# Autodesk Inventor assembly: Front Hitch Model-2
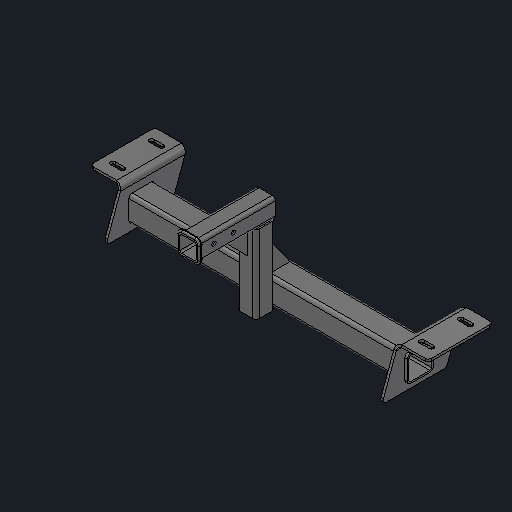
[picture p0: Inventor's stored thumbnail of the model, 512x512]
Saved by Autodesk Inventor 2025.1 (Build 291241000, 241)
## iProperties
Created: 2026-02-13
Part Number: Front Hitch Model-2
Document SubType Name: Assembly
Designer: Desktop -24
encoded128: ÌStandard (in)rÎ
Family: ASSEMBLY
Author: Desktop -24
## Documents named in this file (8)
- F:\OneDrive - nLeague Technologies Private Limited\Desktop\Sharath Chandra\Front Hitch\Front Hitch Model-2\Front Hitch Model-2.iam
- F:\OneDrive - nLeague Technologies Private Limited\Desktop\Sharath Chandra\Front Hitch\Front Hitch Model-1\Front Hitch Model-1_Base Tube-2.ipt
- F:\OneDrive - nLeague Technologies Private Limited\Desktop\Sharath Chandra\Front Hitch\Front Hitch Model-2\Front Hitch Model-2_Base Tube-1.ipt
- F:\OneDrive - nLeague Technologies Private Limited\Desktop\Sharath Chandra\Front Hitch\Front Hitch Model-2\Front Hitch Model-1_Base Tube-3.ipt
- F:\OneDrive - nLeague Technologies Private Limited\Desktop\Sharath Chandra\Front Hitch\Front Hitch Model-2\Front Hitch Model-2_Sheet Stifferner-1.ipt
- F:\OneDrive - nLeague Technologies Private Limited\Desktop\Sharath Chandra\Front Hitch\Front Hitch Model-2\Front Hitch Model-2_Sheet Stifferner-2.ipt
- F:\OneDrive - nLeague Technologies Private Limited\Desktop\Sharath Chandra\Front Hitch\Front Hitch Model-2\Front Hitch Model-2_Sheet-RH.ipt
- F:\OneDrive - nLeague Technologies Private Limited\Desktop\Sharath Chandra\Front Hitch\Front Hitch Model-2\Front Hitch Model-2_Sheet-LH.ipt
## Components (7 placed, 7 different names)
1. Front Hitch Model-2_Base Tube-1.ipt:1 — Mate:14, Mate:15, Mate:16, Mate:17, Mate:18, Flush:8, Flush:9, Flush:12, Mate:20, Mate:21, Mate:23
2. Front Hitch Model-2_Sheet-LH.ipt:1 — Mate:17, Mate:18, Flush:8
3. Front Hitch Model-2_Sheet-RH.ipt:1 — Mate:15, Mate:16, Flush:9
4. Front Hitch Model-1_Base Tube-2.ipt:1 — Mate:19, Flush:10, Flush:11, Mate:25
5. Front Hitch Model-1_Base Tube-3.ipt:1 — Mate:19, Flush:10, Flush:11, Flush:12, Mate:20, Mate:21, Mate:22, Mate:24
6. Front Hitch Model-2_Sheet Stifferner-2.ipt:1 — Mate:22, Mate:23
7. Front Hitch Model-2_Sheet Stifferner-1.ipt:1 — Mate:24, Mate:25
## Relationships (17: Mate 12, Flush 5)
- Mate:14: Front Hitch Model-2_Base Tube-1.ipt:1
- Mate:15: Front Hitch Model-2_Base Tube-1.ipt:1 ↔ Front Hitch Model-2_Sheet-RH.ipt:1
- Mate:16: Front Hitch Model-2_Base Tube-1.ipt:1 ↔ Front Hitch Model-2_Sheet-RH.ipt:1
- Mate:17: Front Hitch Model-2_Base Tube-1.ipt:1 ↔ Front Hitch Model-2_Sheet-LH.ipt:1
- Mate:18: Front Hitch Model-2_Base Tube-1.ipt:1 ↔ Front Hitch Model-2_Sheet-LH.ipt:1
- Flush:8 (9.525 mm): Front Hitch Model-2_Base Tube-1.ipt:1 ↔ Front Hitch Model-2_Sheet-LH.ipt:1
- Flush:9 (-9.525 mm): Front Hitch Model-2_Base Tube-1.ipt:1 ↔ Front Hitch Model-2_Sheet-RH.ipt:1
- Mate:19: Front Hitch Model-1_Base Tube-2.ipt:1 ↔ Front Hitch Model-1_Base Tube-3.ipt:1
- Flush:10: Front Hitch Model-1_Base Tube-2.ipt:1 ↔ Front Hitch Model-1_Base Tube-3.ipt:1
- Flush:11: Front Hitch Model-1_Base Tube-2.ipt:1 ↔ Front Hitch Model-1_Base Tube-3.ipt:1
- Flush:12: Front Hitch Model-2_Base Tube-1.ipt:1 ↔ Front Hitch Model-1_Base Tube-3.ipt:1
- Mate:20: Front Hitch Model-2_Base Tube-1.ipt:1 ↔ Front Hitch Model-1_Base Tube-3.ipt:1
- Mate:21: Front Hitch Model-2_Base Tube-1.ipt:1 ↔ Front Hitch Model-1_Base Tube-3.ipt:1
- Mate:22: Front Hitch Model-1_Base Tube-3.ipt:1 ↔ Front Hitch Model-2_Sheet Stifferner-2.ipt:1
- Mate:23: Front Hitch Model-2_Base Tube-1.ipt:1 ↔ Front Hitch Model-2_Sheet Stifferner-2.ipt:1
- Mate:24: Front Hitch Model-1_Base Tube-3.ipt:1 ↔ Front Hitch Model-2_Sheet Stifferner-1.ipt:1
- Mate:25: Front Hitch Model-1_Base Tube-2.ipt:1 ↔ Front Hitch Model-2_Sheet Stifferner-1.ipt:1
